# Autodesk Inventor assembly: PLA_SetCollar_d6
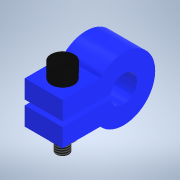
[picture p0: Inventor's stored thumbnail of the model, 180x180]
Saved by Autodesk Inventor 2022 (Build 260153000, 153)
## iProperties
Created: 2020-12-13
Part Number: PLA_SetCollar_d6
Document SubType Name: Assembly
Designer: Hagihara Yuya
Author: Hagihara Yuya
## Documents named in this file (4)
- C:\Users\shiot\OneDrive\ドキュメント\GrabCAD\NHK2022\BasicParts\SetColor\PLA_SetCollar_d6\PLA_SetCollar_d6.iam
- C:\Users\shiot\OneDrive\ドキュメント\GrabCAD\NHK2022\BasicParts\SetColor\PLA_SetCollar_d6\PLA_SetCollar_d6.ipt
- C:\Users\shiot\OneDrive\ドキュメント\GrabCAD\NHK2022\BasicParts\SetColor\PLA_SetCollar_d6\Bolt_M3_15_for_SetCollar_d6.ipt
- C:\Users\shiot\OneDrive\ドキュメント\GrabCAD\NHK2022\BasicParts\SetColor\PLA_SetCollar_d6\Nut_M3_for_SetCollar.ipt
## Components (3 placed, 3 different names)
1. PLA_SetCollar_d6:1 — 回転:1, 回転:2
2. Bolt_M3_15_for_SetCollar_d6:1 — 回転:1
3. Nut_M3_for_SetCollar:1 — 回転:2
## Relationships (2: RevoluteJoint 2)
- 回転:1 [RevoluteJoint]: PLA_SetCollar_d6:1 ↔ Bolt_M3_15_for_SetCollar_d6:1
- 回転:2 [RevoluteJoint]: PLA_SetCollar_d6:1 ↔ Nut_M3_for_SetCollar:1
